# Autodesk Inventor assembly: Sensor_module
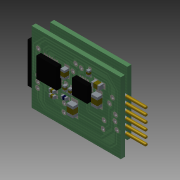
[picture p0: Inventor's stored thumbnail of the model, 180x180]
Saved by Autodesk Inventor 2013 (Build 170138000, 138)
## iProperties
Created: 2015-07-05
Part Number: Sensor_module
Document SubType Name: Assembly
Designer: terg
Author: terg
## Documents named in this file (3)
- C:\Users\terg\Projects\ModularElectronics\3D_models\Sensor_module\Sensor_module.iam
- C:\Users\terg\Projects\ModularElectronics\3D_models\Sensor_module\Sensor_module_envBoard.iam
- C:\Users\terg\Projects\ModularElectronics\3D_models\Sensor_module\Sensor_module_uCMotionBoard.iam
## Components (2 placed, 2 different names)
1. Sensor_module_envBoard:1 [sub-assembly] — Zestawiający:1, Zestawiający:2, Równoległy:1
2. Sensor_module_uCMotionBoard:1 [sub-assembly] — Zestawiający:1, Zestawiający:2, Równoległy:1
## Relationships (3: Mate 2, Flush 1)
- Zestawiający:1 [Mate] (2 mm): Sensor_module_envBoard:1 ↔ Sensor_module_uCMotionBoard:1
- Zestawiający:2 [Mate] (-2.6 mm): Sensor_module_envBoard:1 ↔ Sensor_module_uCMotionBoard:1
- Równoległy:1 [Flush] (0.827 mm): Sensor_module_envBoard:1 ↔ Sensor_module_uCMotionBoard:1
